# Autodesk Inventor assembly: Front Clear Door Assambly
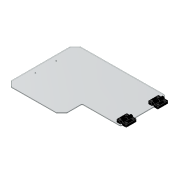
[picture p0: Inventor's stored thumbnail of the model, 180x180]
Saved by Autodesk Inventor 2015 (Build 190159000, 159)
## iProperties
Created: 2018-04-21
Part Number: Front Clear Door Assambly
Document SubType Name: Assembly
Designer: Ghassan Yusuf
Author: Ghassan Yusuf
## Documents named in this file (3)
- X:\Autodesk Designs\MakerBot Transformation\Front Clear Door Assambly.iam
- X:\Autodesk Designs\MakerBot Transformation\Clear Front Door.ipt
- X:\Autodesk Designs\MakerBot Transformation\Hing Assambly.iam
## Components (3 placed, 2 different names)
1. Clear Front Door:1 — Insert:22, Insert:23, Insert:24, Insert:25
2. Hing Assambly:1 [sub-assembly] — Insert:22, Insert:23, Flush:1
3. Hing Assambly:2 [sub-assembly] — Insert:24, Insert:25, Flush:1
## Relationships (5: Insert 4, Flush 1)
- Insert:22: Clear Front Door:1 ↔ Hing Assambly:1
- Insert:23: Clear Front Door:1 ↔ Hing Assambly:1
- Insert:24: Clear Front Door:1 ↔ Hing Assambly:2
- Insert:25: Clear Front Door:1 ↔ Hing Assambly:2
- Flush:1: Hing Assambly:1 ↔ Hing Assambly:2
